# Autodesk Inventor assembly: Robot_6DOF
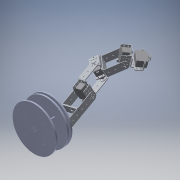
[picture p0: Inventor's stored thumbnail of the model, 180x180]
Saved by Autodesk Inventor 2017 (Build 210142000, 142)
## iProperties
Part Number: Robot_6DOF
Material: Genérico
Document SubType Name: Assembly
Designer: Daniel Caycedo
Author: Daniel Caycedo
## Documents named in this file (7)
- C:\Users\Daniel Caycedo\Documents\Daniel SCR\Universidad\Proyecto ingenieria\Modelo_6R\Inventor\Robot_6DOF.iam
- C:\Users\Daniel Caycedo\Documents\Daniel SCR\Universidad\Proyecto ingenieria\Modelo_6R\Inventor\Base.ipt
- C:\Users\Daniel Caycedo\Documents\Daniel SCR\Universidad\Proyecto ingenieria\Modelo_6R\Inventor\Joint_1.ipt
- C:\Users\Daniel Caycedo\Documents\Daniel SCR\Universidad\Proyecto ingenieria\Modelo_6R\Inventor\Joint_2.ipt
- C:\Users\Daniel Caycedo\Documents\Daniel SCR\Universidad\Proyecto ingenieria\Modelo_6R\Inventor\Joint_3.ipt
- C:\Users\Daniel Caycedo\Documents\Daniel SCR\Universidad\Proyecto ingenieria\Modelo_6R\Inventor\Joint_5.ipt
- C:\Users\Daniel Caycedo\Documents\Daniel SCR\Universidad\Proyecto ingenieria\Modelo_6R\Inventor\Joint_4.ipt
## Components (6 placed, 6 different names)
1. Base:1 — Coincidencia:1, Coincidencia:2
2. Joint_1:1 — Coincidencia:1, Coincidencia:2, Coincidencia:3, Coincidencia:4
3. Joint_2:1 — Coincidencia:3, Coincidencia:4, Coincidencia:5, Coincidencia:6
4. Joint_3:1 — Coincidencia:5, Coincidencia:6, Coincidencia:7, Coincidencia:8
5. Joint_5:1 — Coincidencia:9, Coincidencia:10
6. Joint_4:1 — Coincidencia:7, Coincidencia:8, Coincidencia:9, Coincidencia:10
## Relationships (10: Mate 10)
- Coincidencia:1 [Mate]: Base:1 ↔ Joint_1:1
- Coincidencia:2 [Mate]: Base:1 ↔ Joint_1:1
- Coincidencia:3 [Mate]: Joint_1:1 ↔ Joint_2:1
- Coincidencia:4 [Mate]: Joint_1:1 ↔ Joint_2:1
- Coincidencia:5 [Mate]: Joint_2:1 ↔ Joint_3:1
- Coincidencia:6 [Mate]: Joint_2:1 ↔ Joint_3:1
- Coincidencia:7 [Mate]: Joint_3:1 ↔ Joint_4:1
- Coincidencia:8 [Mate]: Joint_3:1 ↔ Joint_4:1
- Coincidencia:9 [Mate]: Joint_5:1 ↔ Joint_4:1
- Coincidencia:10 [Mate]: Joint_5:1 ↔ Joint_4:1
